# Autodesk Inventor assembly: PCB
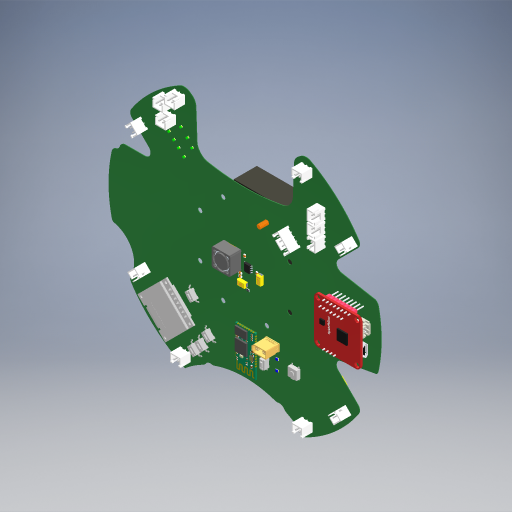
[picture p0: Inventor's stored thumbnail of the model, 512x512]
Saved by Autodesk Inventor 2023 (Build 270158000, 158)
## iProperties
Company: Open CASCADE
Created: 2025-02-04
Part Number: PCB
Description: Open CASCADE Model
Document SubType Name: Assembly
Designer: Ivan
Authority: Unknown
Sending System: Open CASCADE 6.8
Preprocessor: Open CASCADE STEP processor 6.8
Title: Open CASCADE Shape Model
Author: Author
## Documents named in this file (133)
- C:\!projects\DASH-\3D\Dash-V1\0502\PCB1.iam
- C:\!projects\DASH-\3D\Dash-V1\0502\Board.iam
- C:\!projects\DASH-\3D\Dash-V1\0502\R12.iam
- C:\!projects\DASH-\3D\Dash-V1\0502\R11.iam
- C:\!projects\DASH-\3D\Dash-V1\0502\VT2.iam
- C:\!projects\DASH-\3D\Dash-V1\0502\R16.iam
- C:\!projects\DASH-\3D\Dash-V1\0502\D2_2.iam
- C:\!projects\DASH-\3D\Dash-V1\0502\VT1.iam
- C:\!projects\DASH-\3D\Dash-V1\0502\D2_1.iam
- C:\!projects\DASH-\3D\Dash-V1\0502\D1_1.iam
- C:\!projects\DASH-\3D\Dash-V1\0502\+5V.iam
- C:\!projects\DASH-\3D\Dash-V1\0502\+3V3.iam
- C:\!projects\DASH-\3D\Dash-V1\0502\C19.iam
- C:\!projects\DASH-\3D\Dash-V1\0502\C18.iam
- C:\!projects\DASH-\3D\Dash-V1\0502\C13.iam
- C:\!projects\DASH-\3D\Dash-V1\0502\C3_4.iam
- C:\!projects\DASH-\3D\Dash-V1\0502\C3_3.iam
- C:\!projects\DASH-\3D\Dash-V1\0502\C3_2.iam
- C:\!projects\DASH-\3D\Dash-V1\0502\C3_1.iam
- C:\!projects\DASH-\3D\Dash-V1\0502\C2_4.iam
- C:\!projects\DASH-\3D\Dash-V1\0502\C2_3.iam
- C:\!projects\DASH-\3D\Dash-V1\0502\C2_2.iam
- C:\!projects\DASH-\3D\Dash-V1\0502\C2_1.iam
- C:\!projects\DASH-\3D\Dash-V1\0502\C12.iam
- C:\!projects\DASH-\3D\Dash-V1\0502\sen1_power.iam
- C:\!projects\DASH-\3D\Dash-V1\0502\sen2_power.iam
- C:\!projects\DASH-\3D\Dash-V1\0502\sen1.iam
- C:\!projects\DASH-\3D\Dash-V1\0502\sen2.iam
- C:\!projects\DASH-\3D\Dash-V1\0502\dribler_data.iam
- C:\!projects\DASH-\3D\Dash-V1\0502\dribler_power.iam
- C:\!projects\DASH-\3D\Dash-V1\0502\C9.iam
- C:\!projects\DASH-\3D\Dash-V1\0502\C10.iam
- C:\!projects\DASH-\3D\Dash-V1\0502\C11.iam
- C:\!projects\DASH-\3D\Dash-V1\0502\C14.iam
- C:\!projects\DASH-\3D\Dash-V1\0502\C15.iam
- C:\!projects\DASH-\3D\Dash-V1\0502\C16.iam
- C:\!projects\DASH-\3D\Dash-V1\0502\C17.iam
- C:\!projects\DASH-\3D\Dash-V1\0502\C5.iam
- C:\!projects\DASH-\3D\Dash-V1\0502\C6.iam
- C:\!projects\DASH-\3D\Dash-V1\0502\C7.iam
- C:\!projects\DASH-\3D\Dash-V1\0502\C8.iam
- C:\!projects\DASH-\3D\Dash-V1\0502\DA1.iam
- C:\!projects\DASH-\3D\Dash-V1\0502\L1.iam
- C:\!projects\DASH-\3D\Dash-V1\0502\R32.iam
- C:\!projects\DASH-\3D\Dash-V1\0502\R33.iam
- C:\!projects\DASH-\3D\Dash-V1\0502\R34.iam
- C:\!projects\DASH-\3D\Dash-V1\0502\R35.iam
- C:\!projects\DASH-\3D\Dash-V1\0502\R36.iam
- C:\!projects\DASH-\3D\Dash-V1\0502\R37.iam
- C:\!projects\DASH-\3D\Dash-V1\0502\R38.iam
- C:\!projects\DASH-\3D\Dash-V1\0502\R39.iam
- C:\!projects\DASH-\3D\Dash-V1\0502\R40.iam
- C:\!projects\DASH-\3D\Dash-V1\0502\R17.iam
- C:\!projects\DASH-\3D\Dash-V1\0502\R18.iam
- C:\!projects\DASH-\3D\Dash-V1\0502\R19.iam
- C:\!projects\DASH-\3D\Dash-V1\0502\R20.iam
- C:\!projects\DASH-\3D\Dash-V1\0502\R21.iam
- C:\!projects\DASH-\3D\Dash-V1\0502\R22.iam
- C:\!projects\DASH-\3D\Dash-V1\0502\R23.iam
- C:\!projects\DASH-\3D\Dash-V1\0502\R24.iam
- C:\!projects\DASH-\3D\Dash-V1\0502\R25.iam
- C:\!projects\DASH-\3D\Dash-V1\0502\R26.iam
- C:\!projects\DASH-\3D\Dash-V1\0502\R27.iam
- C:\!projects\DASH-\3D\Dash-V1\0502\R28.iam
- C:\!projects\DASH-\3D\Dash-V1\0502\R29.iam
- C:\!projects\DASH-\3D\Dash-V1\0502\R30.iam
- C:\!projects\DASH-\3D\Dash-V1\0502\R31.iam
- C:\!projects\DASH-\3D\Dash-V1\0502\Power.iam
- C:\!projects\DASH-\3D\Dash-V1\0502\Down.iam
- C:\!projects\DASH-\3D\Dash-V1\0502\Reset.iam
- C:\!projects\DASH-\3D\Dash-V1\0502\Enter.iam
- C:\!projects\DASH-\3D\Dash-V1\0502\Up.iam
- C:\!projects\DASH-\3D\Dash-V1\0502\U2.iam
- C:\!projects\DASH-\3D\Dash-V1\0502\VD12.iam
- C:\!projects\DASH-\3D\Dash-V1\0502\+12V.iam
- C:\!projects\DASH-\3D\Dash-V1\0502\Led1.iam
- C:\!projects\DASH-\3D\Dash-V1\0502\Led2.iam
- C:\!projects\DASH-\3D\Dash-V1\0502\Led3.iam
- C:\!projects\DASH-\3D\Dash-V1\0502\Led4.iam
- C:\!projects\DASH-\3D\Dash-V1\0502\VT3.iam
- C:\!projects\DASH-\3D\Dash-V1\0502\VT4.iam
- C:\!projects\DASH-\3D\Dash-V1\0502\VT5.iam
- C:\!projects\DASH-\3D\Dash-V1\0502\X1.iam
- C:\!projects\DASH-\3D\Dash-V1\0502\D2_3.iam
- C:\!projects\DASH-\3D\Dash-V1\0502\D1_3.iam
- C:\!projects\DASH-\3D\Dash-V1\0502\D1_2.iam
- C:\!projects\DASH-\3D\Dash-V1\0502\R9_1.iam
- C:\!projects\DASH-\3D\Dash-V1\0502\R9_2.iam
- C:\!projects\DASH-\3D\Dash-V1\0502\R9_3.iam
- C:\!projects\DASH-\3D\Dash-V1\0502\R9_4.iam
- C:\!projects\DASH-\3D\Dash-V1\0502\R8_1.iam
- C:\!projects\DASH-\3D\Dash-V1\0502\R8_2.iam
- C:\!projects\DASH-\3D\Dash-V1\0502\R8_3.iam
- C:\!projects\DASH-\3D\Dash-V1\0502\R7_1.iam
- C:\!projects\DASH-\3D\Dash-V1\0502\R7_2.iam
- C:\!projects\DASH-\3D\Dash-V1\0502\R7_3.iam
- C:\!projects\DASH-\3D\Dash-V1\0502\R6_1.iam
- C:\!projects\DASH-\3D\Dash-V1\0502\R6_2.iam
- C:\!projects\DASH-\3D\Dash-V1\0502\R6_3.iam
- C:\!projects\DASH-\3D\Dash-V1\0502\Motor4.iam
- C:\!projects\DASH-\3D\Dash-V1\0502\Motor3.iam
- C:\!projects\DASH-\3D\Dash-V1\0502\Motor2.iam
- C:\!projects\DASH-\3D\Dash-V1\0502\Motor1.iam
- C:\!projects\DASH-\3D\Dash-V1\0502\VD3.iam
- C:\!projects\DASH-\3D\Dash-V1\0502\R15.iam
- C:\!projects\DASH-\3D\Dash-V1\0502\R14.iam
- C:\!projects\DASH-\3D\Dash-V1\0502\R13.iam
- C:\!projects\DASH-\3D\Dash-V1\0502\C4.iam
- C:\!projects\DASH-\3D\Dash-V1\0502\Sol2.iam
- C:\!projects\DASH-\3D\Dash-V1\0502\Sol1.iam
- C:\!projects\DASH-\3D\Dash-V1\0502\Cap.iam
- C:\!projects\DASH-\3D\Dash-V1\0502\IRS4427.iam
- C:\!projects\DASH-\3D\Dash-V1\0502\VD2.iam
- C:\!projects\DASH-\3D\Dash-V1\0502\VD1.iam
- C:\!projects\DASH-\3D\Dash-V1\0502\R5.iam
- C:\!projects\DASH-\3D\Dash-V1\0502\R4.iam
- C:\!projects\DASH-\3D\Dash-V1\0502\R3.iam
- C:\!projects\DASH-\3D\Dash-V1\0502\R2.iam
- C:\!projects\DASH-\3D\Dash-V1\0502\R1.iam
- C:\!projects\DASH-\3D\Dash-V1\0502\open_MV.iam
- C:\!projects\DASH-\3D\Dash-V1\0502\R8_4.iam
- C:\!projects\DASH-\3D\Dash-V1\0502\R7_4.iam
- C:\!projects\DASH-\3D\Dash-V1\0502\R6_4.iam
- C:\!projects\DASH-\3D\Dash-V1\0502\D2_4.iam
- C:\!projects\DASH-\3D\Dash-V1\0502\D1_4.iam
- C:\!projects\DASH-\3D\Dash-V1\0502\VD4.iam
- C:\!projects\DASH-\3D\Dash-V1\0502\blu.iam
- C:\!projects\DASH-\3D\Dash-V1\0502\OLED_SPI1.iam
- C:\!projects\DASH-\3D\Dash-V1\0502\IC1.iam
- C:\!projects\DASH-\3D\Dash-V1\0502\HC1.iam
- C:\!projects\DASH-\3D\Dash-V1\0502\C1.iam
- C:\!projects\DASH-\3D\Dash-V1\step\m3_bolt\Spacer Bolts_m3_bn_L5.ipt
- C:\!projects\DASH-\3D\Dash-V1\boost.ipt
## Components (133 placed, 132 different names)
1. Board_2 [sub-assembly] — Вставка:2
2. R12_8 [sub-assembly]
3. R11_10 [sub-assembly]
4. VT2_20 [sub-assembly]
5. R16_22 [sub-assembly]
6. D2_2_35 [sub-assembly]
7. VT1_37 [sub-assembly]
8. D2_1_39 [sub-assembly]
9. D1_1_41 [sub-assembly]
10. +5V_43 [sub-assembly]
11. +3V3_45 [sub-assembly]
12. C19_47 [sub-assembly]
13. C18_49 [sub-assembly]
14. C13_51 [sub-assembly]
15. C3_4_53 [sub-assembly]
16. C3_3_55 [sub-assembly]
17. C3_2_57 [sub-assembly]
18. C3_1_59 [sub-assembly]
19. C2_4_61 [sub-assembly]
20. C2_3_63 [sub-assembly]
21. C2_2_65 [sub-assembly]
22. C2_1_67 [sub-assembly]
23. C12_69 [sub-assembly]
24. sen1_power_71 [sub-assembly]
25. sen2_power_73 [sub-assembly]
26. sen1_75 [sub-assembly]
27. sen2_77 [sub-assembly]
28. dribler_data_79 [sub-assembly]
29. dribler_power_81 [sub-assembly]
30. C9_83 [sub-assembly]
31. C10_85 [sub-assembly]
32. C11_87 [sub-assembly]
33. C14_89 [sub-assembly]
34. C15_91 [sub-assembly]
35. C16_93 [sub-assembly]
36. C17_95 [sub-assembly]
37. C5_97 [sub-assembly]
38. C6_99 [sub-assembly]
39. C7_101 [sub-assembly]
40. C8_103 [sub-assembly]
41. DA1_105 [sub-assembly]
42. L1_107 [sub-assembly]
43. R32_109 [sub-assembly]
44. R33_111 [sub-assembly]
45. R34_113 [sub-assembly]
46. R35_115 [sub-assembly]
47. R36_117 [sub-assembly]
48. R37_119 [sub-assembly]
49. R38_121 [sub-assembly]
50. R39_123 [sub-assembly]
51. R40_125 [sub-assembly]
52. R17_127 [sub-assembly]
53. R18_129 [sub-assembly]
54. R19_131 [sub-assembly]
55. R20_133 [sub-assembly]
56. R21_135 [sub-assembly]
57. R22_137 [sub-assembly]
58. R23_139 [sub-assembly]
59. R24_141 [sub-assembly]
60. R25_143 [sub-assembly]
61. R26_145 [sub-assembly]
62. R27_147 [sub-assembly]
63. R28_149 [sub-assembly]
64. R29_151 [sub-assembly]
65. R30_153 [sub-assembly]
66. R31_155 [sub-assembly]
67. Power_157 [sub-assembly]
68. Down_159 [sub-assembly]
69. Reset_161 [sub-assembly]
70. Enter_163 [sub-assembly]
71. Up_165 [sub-assembly]
72. U2_167 [sub-assembly]
73. VD12_169 [sub-assembly]
74. +12V_171 [sub-assembly]
75. Led1_173 [sub-assembly]
76. Led2_175 [sub-assembly]
77. Led3_177 [sub-assembly]
78. Led4_179 [sub-assembly]
79. VT3_226 [sub-assembly]
80. VT4_228 [sub-assembly]
81. VT5_231 [sub-assembly]
82. X1_236 [sub-assembly]
83. D2_3_249 [sub-assembly]
84. D1_3_251 [sub-assembly]
85. D1_2_253 [sub-assembly]
86. R9_1_255 [sub-assembly]
87. R9_2_257 [sub-assembly]
88. R9_3_259 [sub-assembly]
89. R9_4_261 [sub-assembly]
90. R8_1_263 [sub-assembly]
91. R8_2_265 [sub-assembly]
92. R8_3_267 [sub-assembly]
93. R7_1_269 [sub-assembly]
94. R7_2_271 [sub-assembly]
95. R7_3_273 [sub-assembly]
96. R6_1_275 [sub-assembly]
97. R6_2_277 [sub-assembly]
98. R6_3_279 [sub-assembly]
99. Motor4_281 [sub-assembly]
100. Motor3_283 [sub-assembly]
101. Motor2_285 [sub-assembly]
102. Motor1_287 [sub-assembly]
103. VD3_289 [sub-assembly]
104. R15_291 [sub-assembly]
105. R14_293 [sub-assembly]
106. R13_295 [sub-assembly]
107. C4_297 [sub-assembly]
108. Sol2_299 [sub-assembly]
109. Sol1_301 [sub-assembly]
110. Cap_303 [sub-assembly]
111. IRS4427_305 [sub-assembly]
112. VD2_307 [sub-assembly]
113. VD1_309 [sub-assembly]
114. R5_311 [sub-assembly]
115. R4_313 [sub-assembly]
116. R3_315 [sub-assembly]
117. R2_317 [sub-assembly]
118. R1_319 [sub-assembly]
119. open_MV_321 [sub-assembly]
120. R8_4_323 [sub-assembly]
121. R7_4_325 [sub-assembly]
122. R6_4_327 [sub-assembly]
123. D2_4_340 [sub-assembly]
124. D1_4_342 [sub-assembly]
125. VD4_344 [sub-assembly]
126. blu_346 [sub-assembly]
127. OLED_SPI1_348 [sub-assembly]
128. IC1_350 [sub-assembly]
129. HC1_352 [sub-assembly]
130. C1_354 [sub-assembly]
131. Spacer Bolts_m3_bn_L5:1 — Вставка:1, Вставка:3
132. Spacer Bolts_m3_bn_L5:2 — Вставка:1, Вставка:2
133. boost:1 — Вставка:3
## Relationships (3: Insert 3)
- Вставка:1 [Insert]: Spacer Bolts_m3_bn_L5:1 ↔ Spacer Bolts_m3_bn_L5:2
- Вставка:2 [Insert]: Board_2 ↔ Spacer Bolts_m3_bn_L5:2
- Вставка:3 [Insert]: Spacer Bolts_m3_bn_L5:1 ↔ boost:1
